# Autodesk Inventor assembly: Vergleiche
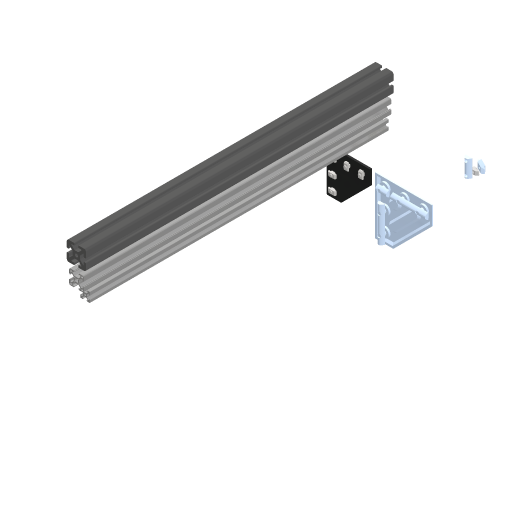
[picture p0: Inventor's stored thumbnail of the model, 512x512]
Saved by Autodesk Inventor 2023 (Build 270158000, 158)
## iProperties
Created: 2024-07-09
Part Number: Vergleiche
Document SubType Name: Assembly
Designer: Nils Bade
Author: Nils Bade
## Documents named in this file (9)
- C:\Users\Nils Bade\Documents\Projektarbeit_Bade\GIT\Masterarbeit-Inventor\Renderings\iams\Vergleiche.iam
- C:\Users\Nils Bade\Documents\Projektarbeit_Bade\GIT\Masterarbeit-Inventor\ITEM\ITEM_0070802_90erKnotenblechsatz 8 40 120x120_MIR.ipt
- C:\Users\Nils Bade\Documents\Projektarbeit_Bade\GIT\Masterarbeit-Inventor\ITEM\4040 Profile\ITEM T-SLOT 4040 640mm.ipt
- C:\Users\Nils Bade\Documents\Projektarbeit_Bade\GIT\Masterarbeit-Inventor\RatRig_Standards\Joining Plate for 3030 Assembly - A v2 (7).iam
- C:\Users\Nils Bade\Documents\Projektarbeit_Bade\GIT\Masterarbeit-Inventor\RatRig_Standards\T-Slot 3030 - Black - 640mm v1.ipt
- C:\Users\Nils Bade\Documents\Projektarbeit_Bade\GIT\Masterarbeit-Inventor\RatRig_Standards\V-Slot 2020 - Black - 622mm v1.ipt
- C:\Users\Nils Bade\Documents\Projektarbeit_Bade\GIT\Masterarbeit-Inventor\ITEM\item_Nutenstein 8 - M3_37359.ipt
- C:\Users\Nils Bade\Documents\Projektarbeit_Bade\GIT\Masterarbeit-Inventor\ITEM\item_Nutenstein 8 - 2xM6-36_0064451.ipt
- C:\Users\Nils Bade\Documents\Projektarbeit_Bade\GIT\Masterarbeit-Inventor\RatRig_modified\T-NUT - DropIn 4040 SERIES - M6.ipt
## Components (8 placed, 8 different names)
1. ITEM_0070802_90erKnotenblechsatz 8 40 120x120_MIR:1 — Fluchtend:3, Passend:7, Fluchtend:4
2. ITEM T-SLOT 4040 640mm:1 — Passend:1, Passend:4, Fluchtend:1, Passend:6
3. Joining Plate for 3030 Assembly - A v2 (7):1 [sub-assembly] — Fluchtend:3, Passend:7, Fluchtend:4
4. T-Slot 3030 - Black - 640mm v1:1 — Passend:2, Passend:4, Passend:5, Fluchtend:1, Fluchtend:2
5. V-Slot 2020 - Black - 622mm v1:1 — Passend:3, Passend:5, Fluchtend:2
6. item_Nutenstein 8 - M3_37359:1 — Passend:8, Passend:11
7. item_Nutenstein 8 - 2xM6-36_0064451:1 — Passend:10, Passend:11, Passend:12
8. T-NUT - DROP IN TYPE FOR 40 SERIES - M6:1 — Passend:9, Passend:12
## Relationships (16: Mate 12, Flush 4)
- Passend:1 [Mate]: ITEM T-SLOT 4040 640mm:1
- Passend:2 [Mate]: T-Slot 3030 - Black - 640mm v1:1
- Passend:3 [Mate]: V-Slot 2020 - Black - 622mm v1:1
- Passend:4 [Mate] (10 mm): ITEM T-SLOT 4040 640mm:1 ↔ T-Slot 3030 - Black - 640mm v1:1
- Passend:5 [Mate] (10 mm): T-Slot 3030 - Black - 640mm v1:1 ↔ V-Slot 2020 - Black - 622mm v1:1
- Fluchtend:1 [Flush]: ITEM T-SLOT 4040 640mm:1 ↔ T-Slot 3030 - Black - 640mm v1:1
- Fluchtend:2 [Flush]: T-Slot 3030 - Black - 640mm v1:1 ↔ V-Slot 2020 - Black - 622mm v1:1
- Passend:6 [Mate]: ITEM T-SLOT 4040 640mm:1
- Fluchtend:3 [Flush]: ITEM_0070802_90erKnotenblechsatz 8 40 120x120_MIR:1 ↔ Joining Plate for 3030 Assembly - A v2 (7):1
- Passend:7 [Mate] (10 mm): ITEM_0070802_90erKnotenblechsatz 8 40 120x120_MIR:1 ↔ Joining Plate for 3030 Assembly - A v2 (7):1
- Fluchtend:4 [Flush]: ITEM_0070802_90erKnotenblechsatz 8 40 120x120_MIR:1 ↔ Joining Plate for 3030 Assembly - A v2 (7):1
- Passend:8 [Mate]: item_Nutenstein 8 - M3_37359:1
- Passend:9 [Mate] (15 mm): T-NUT - DROP IN TYPE FOR 40 SERIES - M6:1
- Passend:10 [Mate] (30 mm): item_Nutenstein 8 - 2xM6-36_0064451:1
- Passend:11 [Mate]: item_Nutenstein 8 - M3_37359:1 ↔ item_Nutenstein 8 - 2xM6-36_0064451:1
- Passend:12 [Mate]: item_Nutenstein 8 - 2xM6-36_0064451:1 ↔ T-NUT - DROP IN TYPE FOR 40 SERIES - M6:1
